# Autodesk Inventor assembly: Bearingandbolts
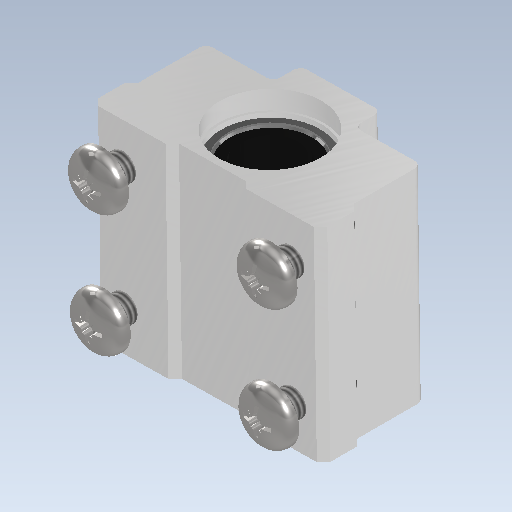
[picture p0: Inventor's stored thumbnail of the model, 512x512]
Saved by Autodesk Inventor 2020.2 (Build 242310000, 310)
## iProperties
Created: 2020-08-25
Part Number: Bearingandbolts
Document SubType Name: Assembly
Designer: JK
Author: JK
## Documents named in this file (3)
- C:\Users\JK\Documents\Inventor\Anet Upgrade\Bearingandbolts.iam
- C:\Users\JK\Documents\Inventor\Anet Upgrade\LinearBearing8mm.iam
- C:\Users\JK\Documents\Inventor\Anet Upgrade\AS 1427 - M4 x 20(6) I.ipt
## Components (5 placed, 2 different names)
1. LinearBearing8mm:1 [sub-assembly] — Mate:1, Mate:2, Mate:3, Mate:4, Mate:5
2. AS 1427 Z - Metryczny M4 x 20:1 — Mate:1, Mate:2, Flush:1, Flush:2
3. AS 1427 Z - Metryczny M4 x 20:2 — Mate:5, Flush:1, Flush:3
4. AS 1427 Z - Metryczny M4 x 20:3 — Mate:4, Flush:2
5. AS 1427 Z - Metryczny M4 x 20:4 — Mate:3, Flush:3
## Relationships (8: Mate 5, Flush 3)
- Mate:1: LinearBearing8mm:1 ↔ AS 1427 Z - Metryczny M4 x 20:1
- Mate:2 (3 mm): LinearBearing8mm:1 ↔ AS 1427 Z - Metryczny M4 x 20:1
- Mate:3: LinearBearing8mm:1 ↔ AS 1427 Z - Metryczny M4 x 20:4
- Mate:4: LinearBearing8mm:1 ↔ AS 1427 Z - Metryczny M4 x 20:3
- Mate:5: LinearBearing8mm:1 ↔ AS 1427 Z - Metryczny M4 x 20:2
- Flush:1: AS 1427 Z - Metryczny M4 x 20:1 ↔ AS 1427 Z - Metryczny M4 x 20:2
- Flush:2: AS 1427 Z - Metryczny M4 x 20:1 ↔ AS 1427 Z - Metryczny M4 x 20:3
- Flush:3: AS 1427 Z - Metryczny M4 x 20:2 ↔ AS 1427 Z - Metryczny M4 x 20:4
